# Autodesk Inventor assembly: Donna2
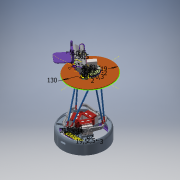
[picture p0: Inventor's stored thumbnail of the model, 180x180]
Saved by Autodesk Inventor 2018.3 (Build 223284000, 284)
## iProperties
Created: 2018-02-24
Part Number: Donna2
Material: Generisch
Document SubType Name: Assembly
Designer: JochenAlt
Author: JochenAlt
## Documents named in this file (6)
- D:\Projects\Donna\CAD\Donna2.iam
- D:\Projects\Donna\CAD\Stewart-Base.iam
- D:\Projects\Donna\CAD\Body-Rod.iam
- D:\Projects\Donna\CAD\Servo-Arm-Head-20mm-Ball-Joint.iam
- D:\Projects\Donna\CAD\PCA9685.ipt
- D:\Projects\Donna\CAD\Head.iam
## Components (15 placed, 5 different names)
1. Stewart-Body:1 [sub-assembly] — Passend:80, Passend:81, Passend:82, Passend:83, Passend:84, Passend:85, Passend:87, Passend:89, Passend:90, Passend:91, Passend:94, Passend:97, Passend:120, Passend:121
2. BodyRod:1 [sub-assembly] — Passend:95, Passend:123
3. BodyRod:2 [sub-assembly] — Passend:96, Passend:122
4. BodyRod:3 [sub-assembly] — Passend:88, Passend:127
5. BodyRod:4 [sub-assembly] — Passend:86, Passend:126
6. BodyRod:5 [sub-assembly] — Passend:93, Passend:125
7. BodyRod:6 [sub-assembly] — Passend:92, Passend:124
8. Servo-Arm-Head-20mm-Ball-Joint:7 [sub-assembly] — Passend:80, Passend:87, Passend:88
9. Servo-Arm-Head-20mm-Ball-Joint:8 [sub-assembly] — Passend:82, Passend:94, Passend:95
10. Servo-Arm-Head-20mm-Ball-Joint:9 [sub-assembly] — Passend:83, Passend:91, Passend:93
11. Servo-Arm-Head-20mm-Ball-Joint:10 [sub-assembly] — Passend:84, Passend:85, Passend:86
12. Servo-Arm-Head-20mm-Ball-Joint:11 [sub-assembly] — Passend:89, Passend:90, Passend:92
13. Servo-Arm-Head-20mm-Ball-Joint:12 [sub-assembly] — Passend:81, Passend:96, Passend:97
14. PCA9685:1 — Passend:120, Passend:121
15. Head:1 [sub-assembly] — Passend:122, Passend:123, Passend:124, Passend:125, Passend:126, Passend:127
## Relationships (26: Mate 26)
- Passend:80 [Mate]: Stewart-Body:1 ↔ Servo-Arm-Head-20mm-Ball-Joint:7
- Passend:81 [Mate]: Stewart-Body:1 ↔ Servo-Arm-Head-20mm-Ball-Joint:12
- Passend:82 [Mate]: Stewart-Body:1 ↔ Servo-Arm-Head-20mm-Ball-Joint:8
- Passend:83 [Mate]: Stewart-Body:1 ↔ Servo-Arm-Head-20mm-Ball-Joint:9
- Passend:84 [Mate]: Stewart-Body:1 ↔ Servo-Arm-Head-20mm-Ball-Joint:10
- Passend:85 [Mate] (2.6 mm): Stewart-Body:1 ↔ Servo-Arm-Head-20mm-Ball-Joint:10
- Passend:86 [Mate]: BodyRod:4 ↔ Servo-Arm-Head-20mm-Ball-Joint:10
- Passend:87 [Mate] (2.6 mm): Stewart-Body:1 ↔ Servo-Arm-Head-20mm-Ball-Joint:7
- Passend:88 [Mate]: BodyRod:3 ↔ Servo-Arm-Head-20mm-Ball-Joint:7
- Passend:89 [Mate]: Stewart-Body:1 ↔ Servo-Arm-Head-20mm-Ball-Joint:11
- Passend:90 [Mate] (2.6 mm): Stewart-Body:1 ↔ Servo-Arm-Head-20mm-Ball-Joint:11
- Passend:91 [Mate] (2.6 mm): Stewart-Body:1 ↔ Servo-Arm-Head-20mm-Ball-Joint:9
- Passend:92 [Mate]: BodyRod:6 ↔ Servo-Arm-Head-20mm-Ball-Joint:11
- Passend:93 [Mate]: BodyRod:5 ↔ Servo-Arm-Head-20mm-Ball-Joint:9
- Passend:94 [Mate] (2.6 mm): Stewart-Body:1 ↔ Servo-Arm-Head-20mm-Ball-Joint:8
- Passend:95 [Mate]: BodyRod:1 ↔ Servo-Arm-Head-20mm-Ball-Joint:8
- Passend:96 [Mate]: BodyRod:2 ↔ Servo-Arm-Head-20mm-Ball-Joint:12
- Passend:97 [Mate] (2.6 mm): Stewart-Body:1 ↔ Servo-Arm-Head-20mm-Ball-Joint:12
- Passend:120 [Mate]: Stewart-Body:1 ↔ PCA9685:1
- Passend:121 [Mate]: Stewart-Body:1 ↔ PCA9685:1
- Passend:122 [Mate]: BodyRod:2 ↔ Head:1
- Passend:123 [Mate]: BodyRod:1 ↔ Head:1
- Passend:124 [Mate]: BodyRod:6 ↔ Head:1
- Passend:125 [Mate]: BodyRod:5 ↔ Head:1
- Passend:126 [Mate]: BodyRod:4 ↔ Head:1
- Passend:127 [Mate]: BodyRod:3 ↔ Head:1
